# Autodesk Inventor assembly: Middle Arm-N
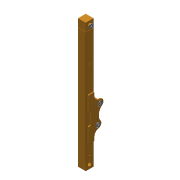
[picture p0: Inventor's stored thumbnail of the model, 180x180]
Saved by Autodesk Inventor 2022 Beta2 (Build 260130000, 130) ContinuousBuild 0
## iProperties
Shininess: 64.0
Length Units: 11269
Angle Units: 11279
Time Units: 11290
Mass Units: 11283
Length Display Precision: 3
Angle Display Precision: 2
Compacted: True
Created: 2003-04-13
Part Number: Middle Arm-N
Document SubType Name: Assembly
Designer: Uffe Bak
Density: 0.0
Volumn: 0.0
Area: 0.0
PropertySet Name: Model Information
Control State: 0
Master: False
Checked Out: False
Author: Uffe Bak
## Documents named in this file (5)
- C:\Autodesk Inventor 2021 Intro Practice Files\BOM\Middle Arm-N.iam
- C:\Autodesk Inventor 2021 Intro Practice Files\BOM\3136 1133 82.iam
- C:\Autodesk Inventor 2021 Intro Practice Files\BOM\3136 7044 74.ipt
- C:\Autodesk Inventor 2021 Intro Practice Files\BOM\3136 7044 79.ipt
- C:\Autodesk Inventor 2021 Intro Practice Files\BOM\3136 7057 14.ipt
## Components (16 placed, 4 different names)
1. 3136 1133 82:1 [sub-assembly] — Insert:26, Insert:27, Insert:28
2. 3136 7044 74:1 — Insert:27, Insert:31, Insert:37
3. 3136 7044 74:2 — Insert:26, Insert:33, Insert:35
4. 3136 7057 14:1 — Insert:34
5. 3136 7044 74:3 — Insert:28, Insert:29, Insert:39
6. 3136 7044 79:3 — Insert:33, Insert:34
7. 3136 7044 79:4 — Insert:31, Insert:32
8. 3136 7044 79:5 — Insert:29, Insert:30
9. 3136 7044 79:6 — Insert:35, Insert:36
10. 3136 7044 79:7 — Insert:37, Insert:38
11. 3136 7044 79:8 — Insert:39, Insert:40
12. 3136 7057 14:3 — Insert:32
13. 3136 7057 14:4 — Insert:30
14. 3136 7057 14:5 — Insert:40
15. 3136 7057 14:6 — Insert:38
16. 3136 7057 14:7 — Insert:36
## Relationships (15: Insert 15)
- Insert:26 (2.25 mm): 3136 1133 82:1 ↔ 3136 7044 74:2
- Insert:27 (2.25 mm): 3136 1133 82:1 ↔ 3136 7044 74:1
- Insert:28 (14.25 mm): 3136 1133 82:1 ↔ 3136 7044 74:3
- Insert:29: 3136 7044 74:3 ↔ 3136 7044 79:5
- Insert:30: 3136 7044 79:5 ↔ 3136 7057 14:4
- Insert:31: 3136 7044 74:1 ↔ 3136 7044 79:4
- Insert:32: 3136 7044 79:4 ↔ 3136 7057 14:3
- Insert:33: 3136 7044 74:2 ↔ 3136 7044 79:3
- Insert:34: 3136 7057 14:1 ↔ 3136 7044 79:3
- Insert:35: 3136 7044 74:2 ↔ 3136 7044 79:6
- Insert:36: 3136 7044 79:6 ↔ 3136 7057 14:7
- Insert:37: 3136 7044 74:1 ↔ 3136 7044 79:7
- Insert:38: 3136 7044 79:7 ↔ 3136 7057 14:6
- Insert:39: 3136 7044 74:3 ↔ 3136 7044 79:8
- Insert:40: 3136 7044 79:8 ↔ 3136 7057 14:5
